# Autodesk Inventor assembly: InternalElectronics
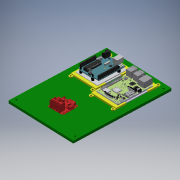
[picture p0: Inventor's stored thumbnail of the model, 180x180]
Saved by Autodesk Inventor 2018 (Build 220112000, 112)
## iProperties
Created: 2018-07-29
Part Number: InternalElectronics
Document SubType Name: Assembly
Designer: jklei
Author: jklei
## Documents named in this file (9)
- C:\Users\jklei\Desktop\Projects\Shamrock\Hardware\Electronics\InternalElectronics.iam
- C:\Users\jklei\Desktop\Projects\Shamrock\Hardware\Electronics\raspberry-pi\raspberry_pi_3_b_plus.iam
- C:\Users\jklei\Desktop\Projects\Shamrock\Hardware\Electronics\Arduino_Uno.ipt
- C:\Users\jklei\Desktop\Projects\Shamrock\Hardware\Electronics\L298N.ipt
- C:\Users\jklei\Desktop\Projects\Shamrock\Hardware\Electronics\pi-holder.ipt
- C:\Users\jklei\Desktop\Projects\Shamrock\Hardware\Electronics\ModBoard-Bottom.ipt
- C:\Users\jklei\Desktop\Projects\Shamrock\Hardware\Electronics\uno-holder.ipt
- C:\Users\jklei\Desktop\Projects\Shamrock\Hardware\Electronics\Electronics-Wedge.ipt
- C:\Users\jklei\Desktop\Projects\Shamrock\Hardware\Electronics\M3-6-6-standoff.ipt
## Components (14 placed, 8 different names)
1. raspberry_pi_3_b_plus:1 [sub-assembly] — Insert:1, Insert:2
2. Arduino_Uno:1 — Insert:10, Angle:1, Insert:11, Insert:12, Insert:13, Angle:2, Angle:3
3. L298N:1
4. pi-holder:1 — Insert:1, Insert:2, Mate:4, Mate:5, Mate:6, Mate:11, Mate:12, Mate:13
5. ModBoard-Bottom:1 — Insert:3, Insert:4, Insert:5, Mate:1
6. uno-holder:1 — Mate:2, Mate:3, Mate:7, Mate:8, Mate:9, Mate:10, Insert:6, Angle:1, Angle:2, Angle:3
7. Electronics-Wedge:1 — Mate:8, Mate:9, Mate:10
8. Electronics-Wedge:2 — Mate:11, Mate:12, Mate:13
9. Electronics-Wedge:3 — Insert:4, Insert:5, Mate:4, Mate:5, Mate:6
10. Electronics-Wedge:4 — Insert:3, Mate:1, Mate:2, Mate:3, Mate:7
11. M3-6-6-standoff:1 — Insert:13
12. M3-6-6-standoff:2 — Insert:12
13. M3-6-6-standoff:3 — Insert:11
14. M3-6-6-standoff:4 — Insert:6, Insert:10
## Relationships (26: Mate 13, Insert 10, Angle 3)
- Insert:1: raspberry_pi_3_b_plus:1 ↔ pi-holder:1
- Insert:2: raspberry_pi_3_b_plus:1 ↔ pi-holder:1
- Insert:3: ModBoard-Bottom:1 ↔ Electronics-Wedge:4
- Insert:4: ModBoard-Bottom:1 ↔ Electronics-Wedge:3
- Insert:5: ModBoard-Bottom:1 ↔ Electronics-Wedge:3
- Mate:1: ModBoard-Bottom:1 ↔ Electronics-Wedge:4
- Mate:2: uno-holder:1 ↔ Electronics-Wedge:4
- Mate:3: uno-holder:1 ↔ Electronics-Wedge:4
- Mate:4: pi-holder:1 ↔ Electronics-Wedge:3
- Mate:5: pi-holder:1 ↔ Electronics-Wedge:3
- Mate:6: pi-holder:1 ↔ Electronics-Wedge:3
- Mate:7: uno-holder:1 ↔ Electronics-Wedge:4
- Mate:8: uno-holder:1 ↔ Electronics-Wedge:1
- Mate:9: uno-holder:1 ↔ Electronics-Wedge:1
- Mate:10: uno-holder:1 ↔ Electronics-Wedge:1
- Mate:11: pi-holder:1 ↔ Electronics-Wedge:2
- Mate:12: pi-holder:1 ↔ Electronics-Wedge:2
- Mate:13: pi-holder:1 ↔ Electronics-Wedge:2
- Insert:6: uno-holder:1 ↔ M3-6-6-standoff:4
- Insert:10: Arduino_Uno:1 ↔ M3-6-6-standoff:4
- Angle:1 (0 deg): Arduino_Uno:1 ↔ uno-holder:1
- Insert:11: Arduino_Uno:1 ↔ M3-6-6-standoff:3
- Insert:12: Arduino_Uno:1 ↔ M3-6-6-standoff:2
- Insert:13: Arduino_Uno:1 ↔ M3-6-6-standoff:1
- Angle:2 (0 deg): Arduino_Uno:1 ↔ uno-holder:1
- Angle:3 (0 deg): Arduino_Uno:1 ↔ uno-holder:1
